# Autodesk Inventor assembly: Arm 1.1
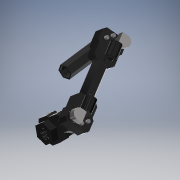
[picture p0: Inventor's stored thumbnail of the model, 180x180]
Saved by Autodesk Inventor 2017 SP1 (Build 210196100, 196)
## iProperties
Created: 2019-09-19
Part Number: Arm 1.1
Document SubType Name: Assembly
Designer: Dell
Author: Dell
## Documents named in this file (4)
- C:\Users\Zach\Documents\GitHub\tr2\Arm 1.1\Arm 1.1.iam
- C:\Users\Zach\Documents\GitHub\tr2\Arm 1.1\A01.ipt
- C:\Users\Zach\Documents\GitHub\tr2\Arm 1.1\A02.ipt
- C:\Users\Zach\Documents\GitHub\tr2\Actuator 2.0\Actuator 2.0.iam
## Components (5 placed, 3 different names)
1. A01:1 — Mate:27, Mate:28, Mate:29, Mate:30, Mate:31, Mate:32, Mate:33
2. A02:1 — Mate:34, Mate:35
3. Actuator 2.0:1 [sub-assembly] — Mate:23, Mate:24, Mate:25, Mate:36
4. Actuator 2.0:2 [sub-assembly] — Mate:25, Mate:27, Mate:28, Mate:29, Mate:36
5. Actuator 2.0:3 [sub-assembly] — Mate:30, Mate:31, Mate:32, Mate:33, Mate:34, Mate:35
## Relationships (13: Mate 13)
- Mate:23: Actuator 2.0:1
- Mate:24: Actuator 2.0:1
- Mate:25: Actuator 2.0:1 ↔ Actuator 2.0:2
- Mate:27: A01:1 ↔ Actuator 2.0:2
- Mate:28: A01:1 ↔ Actuator 2.0:2
- Mate:29: A01:1 ↔ Actuator 2.0:2
- Mate:30: A01:1 ↔ Actuator 2.0:3
- Mate:31: A01:1 ↔ Actuator 2.0:3
- Mate:32: A01:1 ↔ Actuator 2.0:3
- Mate:33: A01:1 ↔ Actuator 2.0:3
- Mate:34: A02:1 ↔ Actuator 2.0:3
- Mate:35: A02:1 ↔ Actuator 2.0:3
- Mate:36: Actuator 2.0:1 ↔ Actuator 2.0:2
